# Autodesk Inventor assembly: Zusammenbau
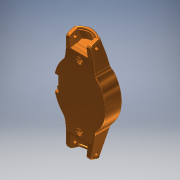
[picture p0: Inventor's stored thumbnail of the model, 180x180]
Saved by Autodesk Inventor 2019 (Build 230136000, 136)
## iProperties
Created: 2021-08-09
Part Number: Zusammenbau
Material: Generisch
Document SubType Name: Assembly
Designer: Bergi
Author: Bergi
## Documents named in this file (3)
- C:\Users\Bergi\Desktop\3D Sketches\Bulova\V3\Zusammenbau.iam
- C:\Users\Bergi\Desktop\3D Sketches\Bulova\V3\Body.ipt
- C:\Users\Bergi\Desktop\3D Sketches\Bulova\V3\Deckel.ipt
## Components (2 placed, 2 different names)
1. Body:1 — Passend:1, Passend:2, Passend:3
2. Deckel:1 — Passend:1, Passend:2, Passend:3
## Relationships (3: Mate 3)
- Passend:1 [Mate]: Body:1 ↔ Deckel:1
- Passend:2 [Mate]: Body:1 ↔ Deckel:1
- Passend:3 [Mate]: Body:1 ↔ Deckel:1
